# Autodesk Inventor assembly: y-carriage
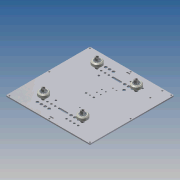
[picture p0: Inventor's stored thumbnail of the model, 180x180]
Saved by Autodesk Inventor 2016 (Build 200138000, 138)
## iProperties
Created: 2015-10-04
Part Number: y-carriage
Document SubType Name: Assembly
Designer: Solomon
Author: Solomon
## Documents named in this file (3)
- C:\Users\Solomon\Documents\Inventor\jonathan-printer\y-carriage.iam
- C:\Users\Solomon\Documents\Inventor\jonathan-printer\V Slot Part Files\V Slot Plates\Universal Build Pate.ipt
- C:\Users\Solomon\Documents\Inventor\jonathan-printer\V Slot Part Files\assembledwheel.iam
## Components (5 placed, 2 different names)
1. Universal Build Pate:1 — Mate:1, Mate:2, Mate:3, Mate:4, Angle:1, Angle:2, Angle:3, Angle:4, Angle:5, Angle:6, Angle:7, Angle:8, Angle:9
2. assembledwheel:1 [sub-assembly] — Mate:1, Angle:3, Angle:8
3. assembledwheel:2 [sub-assembly] — Mate:2, Angle:2, Angle:5
4. assembledwheel:3 [sub-assembly] — Mate:3, Angle:1, Angle:6, Angle:9
5. assembledwheel:4 [sub-assembly] — Mate:4, Angle:4, Angle:7
## Relationships (13: Angle 9, Mate 4)
- Mate:1: Universal Build Pate:1 ↔ assembledwheel:1
- Mate:2: Universal Build Pate:1 ↔ assembledwheel:2
- Mate:3: Universal Build Pate:1 ↔ assembledwheel:3
- Mate:4: Universal Build Pate:1 ↔ assembledwheel:4
- Angle:1 (0 deg): Universal Build Pate:1 ↔ assembledwheel:3
- Angle:2 (0 deg): Universal Build Pate:1 ↔ assembledwheel:2
- Angle:3 (0 deg): Universal Build Pate:1 ↔ assembledwheel:1
- Angle:4 (0 deg): Universal Build Pate:1 ↔ assembledwheel:4
- Angle:5 (0 deg): Universal Build Pate:1 ↔ assembledwheel:2
- Angle:6 (0 deg): Universal Build Pate:1 ↔ assembledwheel:3
- Angle:7 (0 deg): Universal Build Pate:1 ↔ assembledwheel:4
- Angle:8 (0 deg): Universal Build Pate:1 ↔ assembledwheel:1
- Angle:9 (0 deg): Universal Build Pate:1 ↔ assembledwheel:3
